# Autodesk Inventor assembly: halfcut-48t-gear
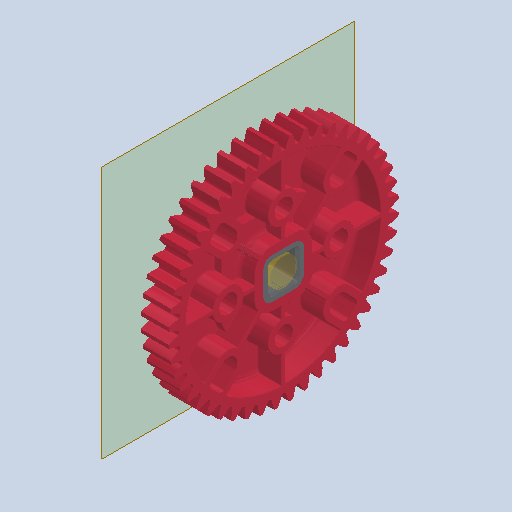
[picture p0: Inventor's stored thumbnail of the model, 512x512]
Saved by Autodesk Inventor 2025.2 (Build 292293000, 293)
## iProperties
Created: 2025-07-20
Part Number: halfcut-48t-gear
Document SubType Name: Assembly
Designer: Exortions
Author: Exortions
## Documents named in this file (3)
- C:\3284b-cad-2025\Library\Custom Parts\halfcut-48t-gear.iam
- C:\3284b-cad-2025\Library\VEX-CAD-Inventor-1.4.2\Motion\Gears\HS Gear\HS 48T Gear, No Insert.iam
- C:\3284b-cad-2025\Library\VEX-CAD-Inventor-1.4.2\Motion\Gears\HS Gear.iam
## Components (1 placed, 1 different names)
1. HS 48T Gear, No Insert:1 [sub-assembly] — Flush:1
## Relationships (1: Flush 1)
- Flush:1: HS 48T Gear, No Insert:1
